# Autodesk Inventor assembly: Bumper Frame
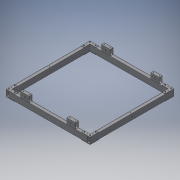
[picture p0: Inventor's stored thumbnail of the model, 180x180]
Saved by Autodesk Inventor 2018 (Build 220112000, 112)
## iProperties
Created: 2019-01-21
Part Number: Bumper Frame
Document SubType Name: Assembly
Designer: maste
Author: maste
## Documents named in this file (7)
- C:\Users\s-2512711\Desktop\Github\2019CAD\Drivebase but Calvin is a mad man\Bumper Frame.iam
- C:\Users\s-2512711\Desktop\Github\2019CAD\Drivebase but Calvin is a mad man\1x1 29in.ipt
- C:\Users\s-2512711\Desktop\Github\2019CAD\Drivebase but Calvin is a mad man\1x1 27in.ipt
- C:\Users\s-2512711\Desktop\Github\2019CAD\Drivebase but Calvin is a mad man\L gusset 2.ipt
- C:\Users\s-2512711\Desktop\Github\2019CAD\Drivebase but Calvin is a mad man\1x1 Bumper Attachment.ipt
- C:\Users\s-2512711\Desktop\Github\2019CAD\Drivebase but Calvin is a mad man\91831A011_TYPE 18-8 STAINLESS STL NYLON-INSERT LOCKNUT.ipt
- C:\Users\s-2512711\Desktop\Github\2019CAD\Drivebase but Calvin is a mad man\73434-Fastenal-01-12-2019.ipt
## Components (40 placed, 6 different names)
1. 1x1 29in:1 — Mate:1, Flush:1, Flush:2, Mate:10, Mate:12, Mate:13, Mate:14, Mate:16, Mate:18, Mate:19, Mate:21
2. 1x1 29in:2 — Mate:2, Flush:3, Flush:4, Mate:3, Flush:5, Flush:6, Mate:4, Mate:5, Mate:7, Mate:9, Mate:24, Mate:26
3. 1x1 27in:1 — Mate:1, Flush:1, Flush:2, Mate:2, Flush:3, Flush:4, Mate:6, Mate:8, Mate:11, Mate:15, Mate:134, Flush:8, Mate:136, Flush:9, Mate:192, Mate:195
4. 1x1 27in:2 — Mate:3, Flush:5, Flush:6, Mate:17, Mate:20, Mate:22, Mate:23, Mate:25, Mate:27, Mate:132, Flush:7, Mate:138, Flush:10, Mate:216
5. L gusset 2:1 — Mate:16, Mate:17, Mate:18, Mate:114, Mate:115, Mate:116
6. L gusset 2:2 — Mate:19, Mate:20, Mate:21, Mate:157, Mate:158, Mate:159, Mate:175, Mate:176, Mate:177
7. L gusset 2:3 — Mate:25, Mate:26, Mate:27, Mate:150, Mate:151, Mate:152, Mate:170, Mate:171, Mate:172
8. L gusset 2:4 — Mate:22, Mate:23, Mate:24, Mate:117, Mate:118, Mate:119
9. L gusset 2:5 — Mate:7, Mate:8, Mate:9, Mate:112, Mate:113
10. L gusset 2:6 — Mate:4, Mate:5, Mate:6, Mate:147, Mate:148, Mate:149, Mate:167, Mate:168, Mate:169
11. L gusset 2:7 — Mate:10, Mate:11, Mate:12, Mate:108, Mate:109, Mate:110
12. L gusset 2:8 — Mate:13, Mate:14, Mate:15, Mate:140, Mate:141, Mate:142, Mate:160, Mate:161, Mate:162
13. 1x1 Bumper Attachment:1 — Mate:132, Flush:7, Mate:216
14. 1x1 Bumper Attachment:2 — Mate:134, Flush:8
15. 1x1 Bumper Attachment:3 — Mate:136, Flush:9, Mate:195
16. 1x1 Bumper Attachment:4 — Mate:138, Flush:10
17. 73434-Fastenal-01-12-2019:8 — Mate:148, Mate:168, Mate:199
18. 91831A011_TYPE 18-8 STAINLESS STL NYLON-INSERT LOCKNUT:1 — Mate:110, Mate:209
19. 91831A011_TYPE 18-8 STAINLESS STL NYLON-INSERT LOCKNUT:2 — Mate:108, Mate:207
20. 91831A011_TYPE 18-8 STAINLESS STL NYLON-INSERT LOCKNUT:3 — Mate:109, Mate:208
21. 91831A011_TYPE 18-8 STAINLESS STL NYLON-INSERT LOCKNUT:4 — Mate:114, Mate:204
22. 91831A011_TYPE 18-8 STAINLESS STL NYLON-INSERT LOCKNUT:5 — Mate:115, Mate:205
23. 91831A011_TYPE 18-8 STAINLESS STL NYLON-INSERT LOCKNUT:6 — Mate:116, Mate:206
24. 91831A011_TYPE 18-8 STAINLESS STL NYLON-INSERT LOCKNUT:7 — Mate:117, Mate:203
25. 91831A011_TYPE 18-8 STAINLESS STL NYLON-INSERT LOCKNUT:8 — Mate:118, Mate:202
26. 91831A011_TYPE 18-8 STAINLESS STL NYLON-INSERT LOCKNUT:9 — Mate:119, Mate:201
27. 91831A011_TYPE 18-8 STAINLESS STL NYLON-INSERT LOCKNUT:10 — Mate:113, Mate:200
28. 91831A011_TYPE 18-8 STAINLESS STL NYLON-INSERT LOCKNUT:11 — Mate:112, Mate:199
29. 73434-Fastenal-01-12-2019:9 — Mate:147, Mate:167, Mate:198
30. 73434-Fastenal-01-12-2019:10 — Mate:149, Mate:169, Mate:200
31. 73434-Fastenal-01-12-2019:11 — Mate:150, Mate:170, Mate:201
32. 73434-Fastenal-01-12-2019:12 — Mate:151, Mate:171, Mate:202
33. 73434-Fastenal-01-12-2019:13 — Mate:152, Mate:172, Mate:203
34. 73434-Fastenal-01-12-2019:14 — Mate:157, Mate:175, Mate:206
35. 73434-Fastenal-01-12-2019:15 — Mate:158, Mate:176, Mate:205
36. 73434-Fastenal-01-12-2019:16 — Mate:159, Mate:177, Mate:204
37. 73434-Fastenal-01-12-2019:17 — Mate:142, Mate:160, Mate:208
38. 73434-Fastenal-01-12-2019:18 — Mate:141, Mate:161, Mate:207
39. 73434-Fastenal-01-12-2019:19 — Mate:140, Mate:162, Mate:209
40. 91831A011_TYPE 18-8 STAINLESS STL NYLON-INSERT LOCKNUT:13 — Mate:192, Mate:198
## Relationships (91: Mate 81, Flush 10)
- Mate:1: 1x1 29in:1 ↔ 1x1 27in:1
- Flush:1: 1x1 29in:1 ↔ 1x1 27in:1
- Flush:2: 1x1 29in:1 ↔ 1x1 27in:1
- Mate:2: 1x1 29in:2 ↔ 1x1 27in:1
- Flush:3: 1x1 29in:2 ↔ 1x1 27in:1
- Flush:4: 1x1 29in:2 ↔ 1x1 27in:1
- Mate:3: 1x1 29in:2 ↔ 1x1 27in:2
- Flush:5: 1x1 29in:2 ↔ 1x1 27in:2
- Flush:6: 1x1 29in:2 ↔ 1x1 27in:2
- Mate:4: 1x1 29in:2 ↔ L gusset 2:6
- Mate:5: 1x1 29in:2 ↔ L gusset 2:6
- Mate:6: 1x1 27in:1 ↔ L gusset 2:6
- Mate:7: 1x1 29in:2 ↔ L gusset 2:5
- Mate:8: 1x1 27in:1 ↔ L gusset 2:5
- Mate:9: 1x1 29in:2 ↔ L gusset 2:5
- Mate:10: 1x1 29in:1 ↔ L gusset 2:7
- Mate:11: 1x1 27in:1 ↔ L gusset 2:7
- Mate:12: 1x1 29in:1 ↔ L gusset 2:7
- Mate:13: 1x1 29in:1 ↔ L gusset 2:8
- Mate:14: 1x1 29in:1 ↔ L gusset 2:8
- Mate:15: 1x1 27in:1 ↔ L gusset 2:8
- Mate:16: 1x1 29in:1 ↔ L gusset 2:1
- Mate:17: 1x1 27in:2 ↔ L gusset 2:1
- Mate:18: 1x1 29in:1 ↔ L gusset 2:1
- Mate:19: 1x1 29in:1 ↔ L gusset 2:2
- Mate:20: 1x1 27in:2 ↔ L gusset 2:2
- Mate:21: 1x1 29in:1 ↔ L gusset 2:2
- Mate:22: 1x1 27in:2 ↔ L gusset 2:4
- Mate:23: 1x1 27in:2 ↔ L gusset 2:4
- Mate:24: 1x1 29in:2 ↔ L gusset 2:4
- Mate:25: 1x1 27in:2 ↔ L gusset 2:3
- Mate:26: 1x1 29in:2 ↔ L gusset 2:3
- Mate:27: 1x1 27in:2 ↔ L gusset 2:3
- Mate:108: L gusset 2:7 ↔ 91831A011_TYPE 18-8 STAINLESS STL NYLON-INSERT LOCKNUT:2
- Mate:109: L gusset 2:7 ↔ 91831A011_TYPE 18-8 STAINLESS STL NYLON-INSERT LOCKNUT:3
- Mate:110: L gusset 2:7 ↔ 91831A011_TYPE 18-8 STAINLESS STL NYLON-INSERT LOCKNUT:1
- Mate:112: L gusset 2:5 ↔ 91831A011_TYPE 18-8 STAINLESS STL NYLON-INSERT LOCKNUT:11
- Mate:113: L gusset 2:5 ↔ 91831A011_TYPE 18-8 STAINLESS STL NYLON-INSERT LOCKNUT:10
- Mate:114: L gusset 2:1 ↔ 91831A011_TYPE 18-8 STAINLESS STL NYLON-INSERT LOCKNUT:4
- Mate:115: L gusset 2:1 ↔ 91831A011_TYPE 18-8 STAINLESS STL NYLON-INSERT LOCKNUT:5
- Mate:116: L gusset 2:1 ↔ 91831A011_TYPE 18-8 STAINLESS STL NYLON-INSERT LOCKNUT:6
- Mate:117: L gusset 2:4 ↔ 91831A011_TYPE 18-8 STAINLESS STL NYLON-INSERT LOCKNUT:7
- Mate:118: L gusset 2:4 ↔ 91831A011_TYPE 18-8 STAINLESS STL NYLON-INSERT LOCKNUT:8
- Mate:119: L gusset 2:4 ↔ 91831A011_TYPE 18-8 STAINLESS STL NYLON-INSERT LOCKNUT:9
- Mate:132: 1x1 27in:2 ↔ 1x1 Bumper Attachment:1
- Flush:7: 1x1 27in:2 ↔ 1x1 Bumper Attachment:1
- Mate:134: 1x1 27in:1 ↔ 1x1 Bumper Attachment:2
- Flush:8: 1x1 27in:1 ↔ 1x1 Bumper Attachment:2
- Mate:136: 1x1 27in:1 ↔ 1x1 Bumper Attachment:3
- Flush:9: 1x1 27in:1 ↔ 1x1 Bumper Attachment:3
- Mate:138: 1x1 27in:2 ↔ 1x1 Bumper Attachment:4
- Flush:10: 1x1 27in:2 ↔ 1x1 Bumper Attachment:4
- Mate:140: L gusset 2:8 ↔ 73434-Fastenal-01-12-2019:19
- Mate:141: L gusset 2:8 ↔ 73434-Fastenal-01-12-2019:18
- Mate:142: L gusset 2:8 ↔ 73434-Fastenal-01-12-2019:17
- Mate:147: L gusset 2:6 ↔ 73434-Fastenal-01-12-2019:9
- Mate:148: L gusset 2:6 ↔ 73434-Fastenal-01-12-2019:8
- Mate:149: L gusset 2:6 ↔ 73434-Fastenal-01-12-2019:10
- Mate:150: L gusset 2:3 ↔ 73434-Fastenal-01-12-2019:11
- Mate:151: L gusset 2:3 ↔ 73434-Fastenal-01-12-2019:12
- Mate:152: L gusset 2:3 ↔ 73434-Fastenal-01-12-2019:13
- Mate:157: L gusset 2:2 ↔ 73434-Fastenal-01-12-2019:14
- Mate:158: L gusset 2:2 ↔ 73434-Fastenal-01-12-2019:15
- Mate:159: L gusset 2:2 ↔ 73434-Fastenal-01-12-2019:16
- Mate:160: L gusset 2:8 ↔ 73434-Fastenal-01-12-2019:17
- Mate:161: L gusset 2:8 ↔ 73434-Fastenal-01-12-2019:18
- Mate:162: L gusset 2:8 ↔ 73434-Fastenal-01-12-2019:19
- Mate:167: L gusset 2:6 ↔ 73434-Fastenal-01-12-2019:9
- Mate:168: L gusset 2:6 ↔ 73434-Fastenal-01-12-2019:8
- Mate:169: L gusset 2:6 ↔ 73434-Fastenal-01-12-2019:10
- Mate:170: L gusset 2:3 ↔ 73434-Fastenal-01-12-2019:11
- Mate:171: L gusset 2:3 ↔ 73434-Fastenal-01-12-2019:12
- Mate:172: L gusset 2:3 ↔ 73434-Fastenal-01-12-2019:13
- Mate:175: L gusset 2:2 ↔ 73434-Fastenal-01-12-2019:14
- Mate:176: L gusset 2:2 ↔ 73434-Fastenal-01-12-2019:15
- Mate:177: L gusset 2:2 ↔ 73434-Fastenal-01-12-2019:16
- Mate:192: 1x1 27in:1 ↔ 91831A011_TYPE 18-8 STAINLESS STL NYLON-INSERT LOCKNUT:13
- Mate:195: 1x1 27in:1 ↔ 1x1 Bumper Attachment:3
- Mate:198: 73434-Fastenal-01-12-2019:9 ↔ 91831A011_TYPE 18-8 STAINLESS STL NYLON-INSERT LOCKNUT:13
- Mate:199: 73434-Fastenal-01-12-2019:8 ↔ 91831A011_TYPE 18-8 STAINLESS STL NYLON-INSERT LOCKNUT:11
- Mate:200: 91831A011_TYPE 18-8 STAINLESS STL NYLON-INSERT LOCKNUT:10 ↔ 73434-Fastenal-01-12-2019:10
- Mate:201: 91831A011_TYPE 18-8 STAINLESS STL NYLON-INSERT LOCKNUT:9 ↔ 73434-Fastenal-01-12-2019:11
- Mate:202: 91831A011_TYPE 18-8 STAINLESS STL NYLON-INSERT LOCKNUT:8 ↔ 73434-Fastenal-01-12-2019:12
- Mate:203: 91831A011_TYPE 18-8 STAINLESS STL NYLON-INSERT LOCKNUT:7 ↔ 73434-Fastenal-01-12-2019:13
- Mate:204: 91831A011_TYPE 18-8 STAINLESS STL NYLON-INSERT LOCKNUT:4 ↔ 73434-Fastenal-01-12-2019:16
- Mate:205: 91831A011_TYPE 18-8 STAINLESS STL NYLON-INSERT LOCKNUT:5 ↔ 73434-Fastenal-01-12-2019:15
- Mate:206: 91831A011_TYPE 18-8 STAINLESS STL NYLON-INSERT LOCKNUT:6 ↔ 73434-Fastenal-01-12-2019:14
- Mate:207: 91831A011_TYPE 18-8 STAINLESS STL NYLON-INSERT LOCKNUT:2 ↔ 73434-Fastenal-01-12-2019:18
- Mate:208: 91831A011_TYPE 18-8 STAINLESS STL NYLON-INSERT LOCKNUT:3 ↔ 73434-Fastenal-01-12-2019:17
- Mate:209: 91831A011_TYPE 18-8 STAINLESS STL NYLON-INSERT LOCKNUT:1 ↔ 73434-Fastenal-01-12-2019:19
- Mate:216: 1x1 27in:2 ↔ 1x1 Bumper Attachment:1
